# Autodesk Inventor assembly: Робот RRO 2021
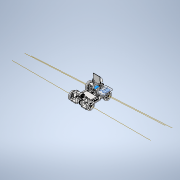
[picture p0: Inventor's stored thumbnail of the model, 180x180]
Saved by Autodesk Inventor 2020 (Build 240168000, 168)
## iProperties
Created: 2021-02-28
Part Number: Робот RRO 2021
Document SubType Name: Assembly
Designer: Антон
Author: Антон
## Documents named in this file (40)
- D:\Project\Robots\FutureEngineersViolet\3D-models\RRO 2021 Mk. III\Робот RRO 2021 Mk. III.iam
- D:\Project\Robots\FutureEngineersViolet\3D-models\RRO 2021 Mk. III\Body\Основа робота.ipt
- D:\Project\Robots\FutureEngineersViolet\3D-models\RRO 2021 Mk. III\Components\Кронштейн для двигателей серии N.ipt
- D:\Project\Robots\FutureEngineersViolet\3D-models\RRO 2021 Mk. III\Components\Servo SG90.ipt
- D:\Project\Robots\FutureEngineersViolet\3D-models\RRO 2021 Mk. III\Body\Основа рулевого механизма.ipt
- D:\Project\Robots\FutureEngineersViolet\3D-models\RRO 2021 Mk. III\Components\Подшипники\Подшипник 3 8 3.ipt
- D:\Project\Robots\FutureEngineersViolet\3D-models\RRO 2021 Mk. III\Components\Оси\Ось 3мм рулевого управления.ipt
- D:\Project\Robots\FutureEngineersViolet\3D-models\RRO 2021 Mk. III\Body\Деталь крепления диска к поворотному механизму.ipt
- D:\Project\Robots\FutureEngineersViolet\3D-models\RRO 2021 Mk. III\Components\Оси\Ось 3мм колеса.ipt
- D:\Project\Robots\FutureEngineersViolet\3D-models\RRO 2021 Mk. III\Body\Деталь крепления диска к поворотному механизму_ЗЕРКАЛО1.ipt
- D:\Project\Robots\FutureEngineersViolet\3D-models\RRO 2021 Mk. III\Components\Micro Gearmotors.ipt
- D:\Project\Robots\FutureEngineersViolet\3D-models\RRO 2021 Mk. III\Body\Стойка для камеры.ipt
- D:\Project\Robots\FutureEngineersViolet\3D-models\RRO 2021 Mk. III\Components\Оси\Ось 2мм рулевой сервы.ipt
- D:\Project\Robots\FutureEngineersViolet\3D-models\RRO 2021 Mk. III\Body\Поворотный рычаг для сервы.ipt
- D:\Project\Robots\FutureEngineersViolet\3D-models\RRO 2021 Mk. III\Body\Крышка стойки подшипника 3мм.ipt
- D:\Project\Robots\FutureEngineersViolet\3D-models\RRO 2021 Mk. III\Body\Съемная стойка сервы.ipt
- D:\Project\Robots\FutureEngineersViolet\3D-models\RRO 2021 Mk. III\Body\Крышка поворотного кулака.ipt
- D:\Project\Robots\FutureEngineersViolet\3D-models\RRO 2021 Mk. III\Body\Стойка подшипника 3мм.ipt
- D:\Project\Robots\FutureEngineersViolet\3D-models\RRO 2021 Mk. III\Components\Оси\Ось 3мм задняя.ipt
- D:\Project\Robots\FutureEngineersViolet\3D-models\RRO 2021 Mk. III\Components\Дифференциал.ipt
- D:\Project\Robots\FutureEngineersViolet\3D-models\RRO 2021 Mk. III\Body\Ведущая шестерня дифференециала.ipt
- D:\Project\Robots\FutureEngineersViolet\3D-models\RRO 2021 Mk. III\Components\Подшипники\Подшипник 10 15 4.ipt
- D:\Project\Robots\FutureEngineersViolet\3D-models\RRO 2021 Mk. III\Body\Переходник с дифференциала на ось 3мм.ipt
- D:\Project\Robots\FutureEngineersViolet\3D-models\RRO 2021 Mk. III\Components\Оси\Ось мотора серии N.ipt
- D:\Project\Robots\FutureEngineersViolet\3D-models\RRO 2021 Mk. III\Body\Крепление дифференциала.ipt
- D:\Project\Robots\FutureEngineersViolet\3D-models\RRO 2021 Mk. III\Body\Крепление двигателя.ipt
- D:\Project\Robots\FutureEngineersViolet\3D-models\RRO 2021 Mk. III\Body\Проставка для двигателя.ipt
- D:\Project\Robots\FutureEngineersViolet\3D-models\RRO 2021 Mk. III\Components\Колесо D40 под ось моторов серии N.ipt
- D:\Project\Robots\FutureEngineersViolet\3D-models\RRO 2021 Mk. III\Body\Деталь основы рулевого управления.ipt
- D:\Project\Robots\FutureEngineersViolet\3D-models\RRO 2021 Mk. III\Body\Крепление USB.ipt
- D:\Project\Robots\FutureEngineersViolet\3D-models\RRO 2021 Mk. III\Body\Крышка USB.ipt
- D:\Project\Robots\FutureEngineersViolet\3D-models\RRO 2021 Mk. III\Components\Подшипники\Подшипник 3 8 4.ipt
- D:\Project\Robots\FutureEngineersViolet\3D-models\RRO 2021 Mk. III\Components\Техническое зрение OpenMV.ipt
- D:\Project\Robots\FutureEngineersViolet\3D-models\RRO 2021 Mk. III\Body\Крепление OpenMV.ipt
- D:\Project\Robots\FutureEngineersViolet\3D-models\RRO 2021 Mk. III\Components\nVision lipo battery.ipt
- D:\Project\Robots\FutureEngineersViolet\3D-models\RRO 2021 Mk. III\Body\Стойка под электроннику.ipt
- D:\Project\Robots\FutureEngineersViolet\3D-models\RRO 2021 Mk. III\Body\Лого ШП.ipt
- D:\Project\Robots\FutureEngineersViolet\3D-models\RRO 2021 Mk. III\Body\Крышка аккумулятора.ipt
- D:\Project\Robots\FutureEngineersViolet\3D-models\RRO 2021 Mk. III\Body\Рулевая тяга правая.ipt
- D:\Project\Robots\FutureEngineersViolet\3D-models\RRO 2021 Mk. III\Body\Рулевая тяга левая.ipt
## Components (63 placed, 38 different names)
1. Основа робота:1 — Жесткий:152, Жесткий:153, Жесткий:189, Жесткий:190, Жесткий:226, Жесткий:231
2. Подшипник 3*8*4:1 — Жесткий:229, С поворотом:167
3. Подшипник 3*8*4:2 — Жесткий:228, С поворотом:166
4. Техническое зрение OpenMV R2:1 — Жесткий:230
5. Крепление OpenMV:1 — Жесткий:230, С поворотом:232
6. nVision lipo battery:1 — Жесткий:234
7. Стойка под электроннику:1 — Жесткий:231, Жесткий:234, Жесткий:241, Жесткий:242
8. Крышка поворотного кулака:3 — Жесткий:239
9. Крышка поворотного кулака:4 — Жесткий:237
10. Лого ШП:1 — Жесткий:241
11. Крышка аккумулятора:1 — Жесткий:242
12. Рулевая тяга правая:1 — С поворотом:249, С поворотом:252
13. Рулевая тяга правая:2 — С поворотом:250, С поворотом:253
14. Стойка для камеры:1 — С поворотом:232, Жесткий:243
15. Основа рулевого механизма:1 — Жесткий:45, Жесткий:226, Жесткий:232, Жесткий:236, Жесткий:238, Жесткий:243, С поворотом:244, С поворотом:248, Жесткий:249, Жесткий:250
16. Съемная стойка сервы:1 — Жесткий:232
17. Поворотный рычаг для сервы:1 — С поворотом:163, С поворотом:252, Жесткий:251
18. Servo SG90:2 — С поворотом:163, Жесткий:238
19. Ось 2мм рулевой сервы:1 — Жесткий:251, С поворотом:253
20. Деталь основы рулевого управления:2 — Жесткий:248, Жесткий:250
21. Деталь основы рулевого управления:1 — Жесткий:223, Жесткий:249
22. Ось 3мм задняя:2 — Жесткий:165, Жесткий:197
23. Крепление двигателя:1 — Жесткий:194, Жесткий:213
24. Переходник с дифференциала на ось 3мм:1 — Жесткий:165, Жесткий:171
25. Дифференциал:1 — С поворотом:158, Жесткий:166, ЗубчПер:1, Жесткий:171, С поворотом:164
26. Переходник с дифференциала на ось 3мм:2 — Жесткий:166, Жесткий:170
27. Ось 3мм задняя:1 — Жесткий:170, Жесткий:196
28. Колесо D40 под ось моторов серии N:1 — Жесткий:196
29. Колесо D40 под ось моторов серии N:2 — Жесткий:199
30. Колесо D40 под ось моторов серии N:4 — Жесткий:197
31. Колесо D40 под ось моторов серии N:3 — Жесткий:198
32. Крышка поворотного кулака:2
33. Деталь крепления диска к поворотному механизму:1 — Жесткий:13, Жесткий:14, Жесткий:229, Жесткий:239, С поворотом:244, С поворотом:250
34. Деталь крепления диска к поворотному механизму_ЗЕРКАЛО1:1 — Жесткий:247, Жесткий:228, Жесткий:237, Жесткий:246, С поворотом:248, С поворотом:249
35. Кронштейн для двигателей серии N:1 — Жесткий:174, Жесткий:193
36. Micro Gearmotors:1 — С поворотом:160, Жесткий:174
37. Проставка для двигателя:1 — Жесткий:193, Жесткий:194
38. Ось мотора серии N:1 — С поворотом:160, Жесткий:192
39. Ведущая шестерня дифференециала:1 — ЗубчПер:1, Жесткий:192
40. Крышка стойки подшипника 3мм:1 — Жесткий:109, Жесткий:110, Жесткий:222
41. Подшипник 3*8*3:9 — Жесткий:109
42. Стойка подшипника 3мм:1 — Жесткий:110, Жесткий:153
43. Крепление USB:1 — Жесткий:220
44. Крышка USB:1 — Жесткий:220, Жесткий:221, Жесткий:222
45. Крепление USB:2 — Жесткий:221
46. Крепление дифференциала:1 — Жесткий:188, Жесткий:189, Жесткий:213
47. Подшипник 10 15 4:1 — С поворотом:158, Жесткий:188
48. Крепление дифференциала:2 — Жесткий:190
49. Подшипник 10 15 4:2 — С поворотом:164
50. Крышка стойки подшипника 3мм:4 — Жесткий:114, Жесткий:163
51. Подшипник 3*8*3:10 — Жесткий:163
52. Стойка подшипника 3мм:4 — Жесткий:114, Жесткий:152
53. Ось 3мм рулевого управления:3 — Жесткий:14
54. Ось 3мм колеса:1 — Жесткий:199, С поворотом:166
55. Ось 3мм рулевого управления:1 — Жесткий:13
56. Подшипник 3*8*3:1
57. Подшипник 3*8*3:2 — Жесткий:45
58. Подшипник 3*8*3:3 — Жесткий:248
59. Ось 3мм колеса:2 — Жесткий:198, С поворотом:167
60. Ось 3мм рулевого управления:4 — Жесткий:247
61. Ось 3мм рулевого управления:5 — Жесткий:246
62. Подшипник 3*8*3:7 — Жесткий:223
63. Подшипник 3*8*3:6 — Жесткий:236
## Relationships (63: WeldJoint 49, RevoluteJoint 13, RelateRotation 1)
- Жесткий:13 [WeldJoint]: Деталь крепления диска к поворотному механизму:1 ↔ Ось 3мм рулевого управления:1
- Жесткий:14 [WeldJoint]: Деталь крепления диска к поворотному механизму:1 ↔ Ось 3мм рулевого управления:3
- Жесткий:45 [WeldJoint]: Основа рулевого механизма:1 ↔ Подшипник 3*8*3:2
- Жесткий:109 [WeldJoint] (-0.05 mm): Крышка стойки подшипника 3мм:1 ↔ Подшипник 3*8*3:9
- Жесткий:110 [WeldJoint]: Крышка стойки подшипника 3мм:1 ↔ Стойка подшипника 3мм:1
- Жесткий:114 [WeldJoint]: Крышка стойки подшипника 3мм:4 ↔ Стойка подшипника 3мм:4
- Жесткий:152 [WeldJoint]: Основа робота:1 ↔ Стойка подшипника 3мм:4
- Жесткий:153 [WeldJoint]: Основа робота:1 ↔ Стойка подшипника 3мм:1
- С поворотом:158 [RevoluteJoint] (-1 mm): Дифференциал:1 ↔ Подшипник 10 15 4:1
- Жесткий:163 [WeldJoint] (-0.05 mm): Крышка стойки подшипника 3мм:4 ↔ Подшипник 3*8*3:10
- Жесткий:165 [WeldJoint]: Ось 3мм задняя:2 ↔ Переходник с дифференциала на ось 3мм:1
- Жесткий:166 [WeldJoint]: Дифференциал:1 ↔ Переходник с дифференциала на ось 3мм:2
- Жесткий:170 [WeldJoint]: Переходник с дифференциала на ось 3мм:2 ↔ Ось 3мм задняя:1
- ЗубчПер:1 [RelateRotation] (2 ul): Дифференциал:1 ↔ Ведущая шестерня дифференециала:1
- С поворотом:160 [RevoluteJoint]: Micro Gearmotors:1 ↔ Ось мотора серии N:1
- Жесткий:171 [WeldJoint]: Переходник с дифференциала на ось 3мм:1 ↔ Дифференциал:1
- Жесткий:174 [WeldJoint]: Кронштейн для двигателей серии N:1 ↔ Micro Gearmotors:1
- С поворотом:163 [RevoluteJoint] (2 mm): Поворотный рычаг для сервы:1 ↔ Servo SG90:2
- Жесткий:188 [WeldJoint]: Крепление дифференциала:1 ↔ Подшипник 10 15 4:1
- С поворотом:164 [RevoluteJoint] (-1 mm): Дифференциал:1 ↔ Подшипник 10 15 4:2
- Жесткий:189 [WeldJoint]: Основа робота:1 ↔ Крепление дифференциала:1
- Жесткий:190 [WeldJoint]: Основа робота:1 ↔ Крепление дифференциала:2
- Жесткий:192 [WeldJoint]: Ось мотора серии N:1 ↔ Ведущая шестерня дифференециала:1
- Жесткий:193 [WeldJoint]: Кронштейн для двигателей серии N:1 ↔ Проставка для двигателя:1
- Жесткий:194 [WeldJoint]: Крепление двигателя:1 ↔ Проставка для двигателя:1
- Жесткий:196 [WeldJoint]: Ось 3мм задняя:1 ↔ Колесо D40 под ось моторов серии N:1
- Жесткий:197 [WeldJoint]: Ось 3мм задняя:2 ↔ Колесо D40 под ось моторов серии N:4
- Жесткий:198 [WeldJoint]: Колесо D40 под ось моторов серии N:3 ↔ Ось 3мм колеса:2
- Жесткий:199 [WeldJoint]: Колесо D40 под ось моторов серии N:2 ↔ Ось 3мм колеса:1
- Жесткий:213 [WeldJoint]: Крепление двигателя:1 ↔ Крепление дифференциала:1
- Жесткий:220 [WeldJoint]: Крепление USB:1 ↔ Крышка USB:1
- Жесткий:221 [WeldJoint]: Крышка USB:1 ↔ Крепление USB:2
- Жесткий:222 [WeldJoint]: Крышка стойки подшипника 3мм:1 ↔ Крышка USB:1
- Жесткий:223 [WeldJoint]: Деталь основы рулевого управления:1 ↔ Подшипник 3*8*3:7
- Жесткий:247 [WeldJoint]: Деталь крепления диска к поворотному механизму_ЗЕРКАЛО1:1 ↔ Ось 3мм рулевого управления:4
- Жесткий:226 [WeldJoint]: Основа робота:1 ↔ Основа рулевого механизма:1
- Жесткий:228 [WeldJoint]: Подшипник 3*8*4:2 ↔ Деталь крепления диска к поворотному механизму_ЗЕРКАЛО1:1
- С поворотом:166 [RevoluteJoint]: Подшипник 3*8*4:2 ↔ Ось 3мм колеса:1
- Жесткий:229 [WeldJoint]: Подшипник 3*8*4:1 ↔ Деталь крепления диска к поворотному механизму:1
- С поворотом:167 [RevoluteJoint]: Подшипник 3*8*4:1 ↔ Ось 3мм колеса:2
- Жесткий:230 [WeldJoint]: Техническое зрение OpenMV R2:1 ↔ Крепление OpenMV:1
- С поворотом:232 [RevoluteJoint] (0.15 mm): Крепление OpenMV:1 ↔ Стойка для камеры:1
- Жесткий:231 [WeldJoint]: Основа робота:1 ↔ Стойка под электроннику:1
- Жесткий:232 [WeldJoint]: Основа рулевого механизма:1 ↔ Съемная стойка сервы:1
- Жесткий:234 [WeldJoint]: nVision lipo battery:1 ↔ Стойка под электроннику:1
- Жесткий:236 [WeldJoint]: Основа рулевого механизма:1 ↔ Подшипник 3*8*3:6
- Жесткий:237 [WeldJoint]: Крышка поворотного кулака:4 ↔ Деталь крепления диска к поворотному механизму_ЗЕРКАЛО1:1
- Жесткий:238 [WeldJoint]: Основа рулевого механизма:1 ↔ Servo SG90:2
- Жесткий:239 [WeldJoint]: Крышка поворотного кулака:3 ↔ Деталь крепления диска к поворотному механизму:1
- Жесткий:241 [WeldJoint]: Стойка под электроннику:1 ↔ Лого ШП:1
- Жесткий:242 [WeldJoint] (0.1 mm): Стойка под электроннику:1 ↔ Крышка аккумулятора:1
- Жесткий:243 [WeldJoint] (-0.15 mm): Стойка для камеры:1 ↔ Основа рулевого механизма:1
- С поворотом:244 [RevoluteJoint] (0.8 mm): Основа рулевого механизма:1 ↔ Деталь крепления диска к поворотному механизму:1
- Жесткий:246 [WeldJoint]: Деталь крепления диска к поворотному механизму_ЗЕРКАЛО1:1 ↔ Ось 3мм рулевого управления:5
- С поворотом:248 [RevoluteJoint] (0.8 mm): Основа рулевого механизма:1 ↔ Деталь крепления диска к поворотному механизму_ЗЕРКАЛО1:1
- Жесткий:248 [WeldJoint]: Деталь основы рулевого управления:2 ↔ Подшипник 3*8*3:3
- Жесткий:249 [WeldJoint]: Основа рулевого механизма:1 ↔ Деталь основы рулевого управления:1
- Жесткий:250 [WeldJoint]: Основа рулевого механизма:1 ↔ Деталь основы рулевого управления:2
- С поворотом:249 [RevoluteJoint] (0.5 mm): Рулевая тяга правая:1 ↔ Деталь крепления диска к поворотному механизму_ЗЕРКАЛО1:1
- С поворотом:250 [RevoluteJoint] (-0.5 mm): Рулевая тяга правая:2 ↔ Деталь крепления диска к поворотному механизму:1
- С поворотом:252 [RevoluteJoint] (0.5 mm): Рулевая тяга правая:1 ↔ Поворотный рычаг для сервы:1
- Жесткий:251 [WeldJoint]: Поворотный рычаг для сервы:1 ↔ Ось 2мм рулевой сервы:1
- С поворотом:253 [RevoluteJoint]: Рулевая тяга правая:2 ↔ Ось 2мм рулевой сервы:1
